# Autodesk Inventor assembly: aaa_0011_wheel
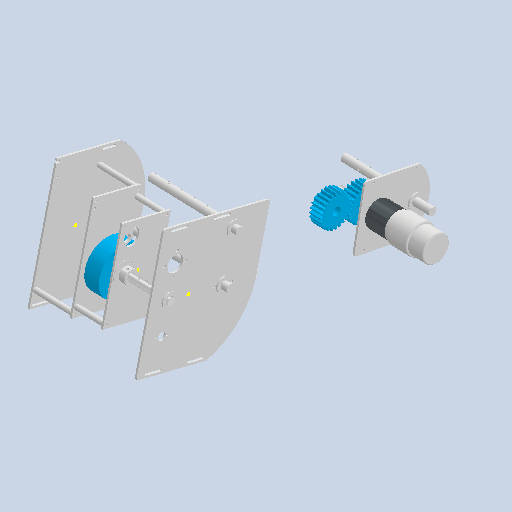
[picture p0: Inventor's stored thumbnail of the model, 512x512]
Saved by Autodesk Inventor 2025.2 (Build 292293000, 293)
## iProperties
Created: 2024-10-03
Part Number: aaa_0011_wheel
Document SubType Name: Assembly
Designer: yuki0520
Author: yuki0520
## Documents named in this file (19)
- C:\Users\haruy\Documents\ロボコン\NHK2025\cad\nagahisa\tanaka_dribll\2025_nhk\tanaka\drible\aaa_0011_wheel.iam
- C:\Users\haruy\Documents\ロボコン\NHK2025\cad\nagahisa\tanaka_dribll\2025_nhk\tanaka\nageru\inventorパーツリスト\モーター\775\RS-775GM.ipt
- C:\Users\haruy\Documents\ロボコン\NHK2025\cad\nagahisa\tanaka_dribll\2025_nhk\tanaka\nageru\inventorパーツリスト\モーター\775\RS-775GM_004GH_sn.ipt
- C:\Users\haruy\Documents\ロボコン\NHK2025\cad\nagahisa\tanaka_dribll\2025_nhk\tanaka\nageru\pakuriz\bear_12_18.ipt
- C:\Users\haruy\Documents\ロボコン\NHK2025\cad\nagahisa\tanaka_dribll\2025_nhk\tanaka\nageru\smallring\small_tire.ipt
- C:\Users\haruy\Documents\ロボコン\NHK2025\cad\nagahisa\tanaka_dribll\2025_nhk\tanaka\nageru\smallring\small_tire_fixer.ipt
- C:\Users\haruy\Documents\ロボコン\NHK2025\cad\nagahisa\tanaka_dribll\2025_nhk\tanaka\nageru\smallring\small_bar_roller.ipt
- C:\Users\haruy\Documents\ロボコン\NHK2025\cad\nagahisa\tanaka_dribll\2025_nhk\tanaka\nageru\smallring\small_gear_motor_48.iam
- C:\Users\haruy\Documents\ロボコン\NHK2025\cad\nagahisa\tanaka_dribll\2025_nhk\tanaka\nageru\smallring\small_bar_motor.ipt
- C:\Users\haruy\Documents\ロボコン\NHK2025\cad\nagahisa\tanaka_dribll\2025_nhk\tanaka\drible\aaa_small_plate_motor.ipt
- C:\Users\haruy\Documents\ロボコン\NHK2025\cad\nagahisa\tanaka_dribll\2025_nhk\tanaka\drible\aaa_small_plate_middle.ipt
- C:\Users\haruy\Documents\ロボコン\NHK2025\cad\nagahisa\tanaka_dribll\2025_nhk\tanaka\drible\aaa_small_plate_no.ipt
- C:\Users\haruy\Documents\ロボコン\NHK2025\cad\nagahisa\tanaka_dribll\2025_nhk\tanaka\drible\aaa_small_plate_arm.ipt
- C:\Users\haruy\Documents\ロボコン\NHK2025\cad\nagahisa\tanaka_dribll\2025_nhk\tanaka\drible\aaa_12_pole.ipt
- C:\Users\haruy\Documents\ロボコン\NHK2025\cad\nagahisa\tanaka_dribll\2025_nhk\tanaka\drible\aaa_gear.iam
- C:\Users\haruy\Documents\ロボコン\NHK2025\cad\nagahisa\tanaka_dribll\2025_nhk\tanaka\drible\aaa_48space.ipt
- C:\Users\haruy\Documents\ロボコン\NHK2025\cad\nagahisa\tanaka_dribll\2025_nhk\tanaka\drible\aaa_64space.ipt
- C:\Users\haruy\Documents\ロボコン\NHK2025\cad\nagahisa\tanaka_dribll\2025_nhk\tanaka\drible\aaa_plate_motor.ipt
- C:\Users\haruy\Documents\ロボコン\NHK2025\cad\nagahisa\tanaka_dribll\2025_nhk\tanaka\drible\aaa_12_jiku_nhisa.ipt
## Components (30 placed, 18 different names)
1. RS-775GM:1 — メイト:4, 正接:1
2. RS-775GM_004GH_sn:1 — メイト:4, 正接:1, メイト:128, メイト:129, メイト:132, 挿入:110, 挿入:111
3. bear_12_18:1 — メイト:33, メイト:116
4. bear_12_18:2 — メイト:35, メイト:110
5. bear_12_18:3 — メイト:31
6. small_tire:1 — メイト:8, 挿入:97, 挿入:98
7. small_tire_fixer:1 — メイト:9
8. small_bar_roller:1 — メイト:8, メイト:9, メイト:30, メイト:31, メイト:33, メイト:35, メイト:88, メイト:96, メイト:102, メイト:111
9. small_tire_fixer:2 — メイト:30, 挿入:97, 挿入:98
10. bear_12_18:4 — メイト:88, メイト:109
11. bear_12_18:5 — メイト:106
12. small_bar_motor:1 — メイト:128, メイト:129, メイト:130, メイト:131
13. aaa_small_plate_motor:1 — メイト:96, メイト:110, メイト:118, メイト:122, 挿入:103, メイト:126, メイト:137, メイト:138, フラッシュ:2
14. aaa_small_plate_middle:1 — メイト:102, メイト:106, メイト:109, 挿入:106, 挿入:108
15. aaa_small_plate_no:1 — メイト:111, メイト:116, 挿入:104, 挿入:105, 挿入:107, 挿入:109
16. aaa_small_plate_arm:1 — メイト:118, メイト:125, 挿入:112, 挿入:113
17. aaa_12_pole:1 — メイト:122, メイト:123, メイト:124, メイト:127
18. aaa_gear:1 [sub-assembly] — メイト:123, 挿入:103
19. bear_12_18:6 — メイト:126, メイト:127
20. bear_12_18:7 — メイト:124, メイト:125
21. aaa_48space:1 — 挿入:107, 挿入:108
22. aaa_48space:2 — 挿入:105, 挿入:106
23. aaa_64space:1 — 挿入:109, 挿入:113
24. aaa_64space:2 — 挿入:104, 挿入:112
25. small_gear_motor_48:1 [sub-assembly] — メイト:130, メイト:131
26. aaa_plate_motor:1 — メイト:132, 挿入:110, 挿入:111, メイト:133, メイト:134, フラッシュ:1
27. bear_12_18:8 — メイト:133, メイト:134, メイト:135
28. aaa_12_jiku_nhisa:1 — メイト:135, フラッシュ:1
29. bear_12_18:9 — メイト:138
30. aaa_12_jiku_nhisa:2 — メイト:137, フラッシュ:2
## Relationships (49: Mate 33, Insert 13, Flush 2, Tangent 1)
- メイト:4 [Mate]: RS-775GM:1 ↔ RS-775GM_004GH_sn:1
- 正接:1 [Tangent]: RS-775GM:1 ↔ RS-775GM_004GH_sn:1
- メイト:8 [Mate]: small_tire:1 ↔ small_bar_roller:1
- メイト:9 [Mate]: small_tire_fixer:1 ↔ small_bar_roller:1
- メイト:30 [Mate]: small_bar_roller:1 ↔ small_tire_fixer:2
- メイト:31 [Mate]: bear_12_18:3 ↔ small_bar_roller:1
- メイト:33 [Mate]: bear_12_18:1 ↔ small_bar_roller:1
- メイト:35 [Mate]: bear_12_18:2 ↔ small_bar_roller:1
- メイト:88 [Mate]: small_bar_roller:1 ↔ bear_12_18:4
- 挿入:97 [Insert]: small_tire:1 ↔ small_tire_fixer:2
- 挿入:98 [Insert]: small_tire:1 ↔ small_tire_fixer:2
- メイト:96 [Mate]: small_bar_roller:1 ↔ aaa_small_plate_motor:1
- メイト:102 [Mate]: small_bar_roller:1 ↔ aaa_small_plate_middle:1
- メイト:106 [Mate]: bear_12_18:5 ↔ aaa_small_plate_middle:1
- メイト:109 [Mate]: bear_12_18:4 ↔ aaa_small_plate_middle:1
- メイト:110 [Mate]: bear_12_18:2 ↔ aaa_small_plate_motor:1
- メイト:111 [Mate]: small_bar_roller:1 ↔ aaa_small_plate_no:1
- メイト:116 [Mate]: bear_12_18:1 ↔ aaa_small_plate_no:1
- メイト:118 [Mate]: aaa_small_plate_motor:1 ↔ aaa_small_plate_arm:1
- メイト:122 [Mate]: aaa_small_plate_motor:1 ↔ aaa_12_pole:1
- メイト:123 [Mate]: aaa_12_pole:1 ↔ aaa_gear:1
- 挿入:103 [Insert]: aaa_small_plate_motor:1 ↔ aaa_gear:1
- メイト:124 [Mate]: aaa_12_pole:1 ↔ bear_12_18:7
- メイト:125 [Mate]: aaa_small_plate_arm:1 ↔ bear_12_18:7
- メイト:126 [Mate]: aaa_small_plate_motor:1 ↔ bear_12_18:6
- メイト:127 [Mate]: aaa_12_pole:1 ↔ bear_12_18:6
- 挿入:104 [Insert]: aaa_small_plate_no:1 ↔ aaa_64space:2
- 挿入:105 [Insert]: aaa_small_plate_no:1 ↔ aaa_48space:2
- 挿入:106 [Insert]: aaa_small_plate_middle:1 ↔ aaa_48space:2
- 挿入:107 [Insert]: aaa_small_plate_no:1 ↔ aaa_48space:1
- 挿入:108 [Insert]: aaa_small_plate_middle:1 ↔ aaa_48space:1
- 挿入:109 [Insert]: aaa_small_plate_no:1 ↔ aaa_64space:1
- メイト:128 [Mate]: RS-775GM_004GH_sn:1 ↔ small_bar_motor:1
- メイト:129 [Mate]: RS-775GM_004GH_sn:1 ↔ small_bar_motor:1
- メイト:130 [Mate]: small_bar_motor:1 ↔ small_gear_motor_48:1
- メイト:131 [Mate]: small_bar_motor:1 ↔ small_gear_motor_48:1
- メイト:132 [Mate]: RS-775GM_004GH_sn:1 ↔ aaa_plate_motor:1
- 挿入:110 [Insert]: RS-775GM_004GH_sn:1 ↔ aaa_plate_motor:1
- 挿入:111 [Insert]: RS-775GM_004GH_sn:1 ↔ aaa_plate_motor:1
- メイト:133 [Mate]: aaa_plate_motor:1 ↔ bear_12_18:8
- メイト:134 [Mate]: aaa_plate_motor:1 ↔ bear_12_18:8
- メイト:135 [Mate]: bear_12_18:8 ↔ aaa_12_jiku_nhisa:1
- フラッシュ:1 [Flush] (-30 mm): aaa_plate_motor:1 ↔ aaa_12_jiku_nhisa:1
- 挿入:112 [Insert]: aaa_small_plate_arm:1 ↔ aaa_64space:2
- 挿入:113 [Insert]: aaa_small_plate_arm:1 ↔ aaa_64space:1
- [Mate]: bear_12_18:9 ↔ aaa_12_jiku_nhisa:2
- メイト:137 [Mate]: aaa_small_plate_motor:1 ↔ aaa_12_jiku_nhisa:2
- メイト:138 [Mate]: aaa_small_plate_motor:1 ↔ bear_12_18:9
- フラッシュ:2 [Flush] (-10 mm): aaa_small_plate_motor:1 ↔ aaa_12_jiku_nhisa:2
## Named parameters: d297_d291 = 0 mm
